# Autodesk Inventor assembly: outerspinner assembled
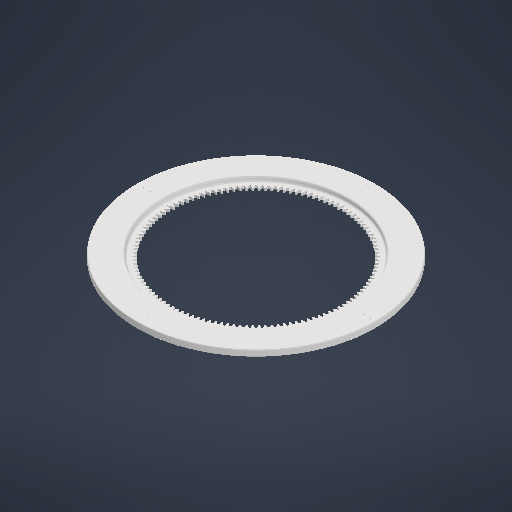
[picture p0: Inventor's stored thumbnail of the model, 512x512]
Saved by Autodesk Inventor 2026 (Build 300175050, 175E)
## iProperties
Created: 2026-05-08
Part Number: outerspinner assembled
Document SubType Name: Assembly
Designer: sniel
Author: sniel
## Documents named in this file (2)
- C:\Users\sniel\OneDrive\SDU\4_Semester\Applied automation\AppliedAutomationProject\feeder\trayFeeder\outerspinner assembled.iam
- C:\Users\sniel\OneDrive\SDU\4_Semester\Applied automation\AppliedAutomationProject\feeder\outerspinner_v3.ipt
## Components (4 placed, 1 different names)
1. outerspinner_v3:1 — Mate:1, Mate:2, Mate:7
2. outerspinner_v3:2 — Mate:1, Mate:2, Mate:3, Mate:4
3. outerspinner_v3:3 — Mate:3, Mate:4, Mate:5, Mate:6
4. outerspinner_v3:4 — Mate:5, Mate:6, Mate:7
## Relationships (7: Mate 7)
- Mate:1: outerspinner_v3:1 ↔ outerspinner_v3:2
- Mate:2: outerspinner_v3:1 ↔ outerspinner_v3:2
- Mate:3: outerspinner_v3:2 ↔ outerspinner_v3:3
- Mate:4: outerspinner_v3:2 ↔ outerspinner_v3:3
- Mate:5: outerspinner_v3:3 ↔ outerspinner_v3:4
- Mate:6: outerspinner_v3:3 ↔ outerspinner_v3:4
- Mate:7: outerspinner_v3:1 ↔ outerspinner_v3:4
